# Autodesk Inventor assembly: A2017_T3_01
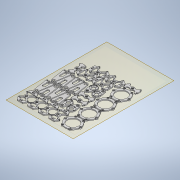
[picture p0: Inventor's stored thumbnail of the model, 180x180]
Saved by Autodesk Inventor 2020 (Build 240168000, 168)
## iProperties
Created: 2021-08-27
Part Number: A2017_T3_01
Document SubType Name: Assembly
Designer: Masato
Author: Masato
## Documents named in this file (7)
- C:\Users\naoki\Documents\Inventor\CitBrains\git_clone\SUSTAINA_ver1_0\A2017_T5_02(sustaina_op)\SUSTAINA-OP\Cam\A2017_T3_01.iam
- C:\Users\naoki\Documents\Inventor\CitBrains\git_clone\SUSTAINA_ver1_0\A2017_T5_02(sustaina_op)\SUSTAINA-OP\Cam\DisposableBoard.ipt
- C:\Users\naoki\Documents\Inventor\CitBrains\git_clone\SUSTAINA_ver1_0\A2017_T5_02(sustaina_op)\SUSTAINA-OP\LowerBody\Leg_joit\Leg_joint_roll_frame.ipt
- C:\Users\naoki\Documents\Inventor\CitBrains\git_clone\SUSTAINA_ver1_0\A2017_T5_02(sustaina_op)\SUSTAINA-OP\LowerBody\Leg_joit\Leg_joint_slider_frame.ipt
- C:\Users\naoki\Documents\Inventor\CitBrains\git_clone\SUSTAINA_ver1_0\A2017_T5_02(sustaina_op)\SUSTAINA-OP\LowerBody\Slider_crank\Slider_crank_horn.ipt
- C:\Users\naoki\Documents\Inventor\CitBrains\git_clone\SUSTAINA_ver1_0\A2017_T5_02(sustaina_op)\SUSTAINA-OP\LowerBody\Ankle\Ankle_front_frame.ipt
- C:\Users\naoki\Documents\Inventor\CitBrains\git_clone\SUSTAINA_ver1_0\A2017_T5_02(sustaina_op)\SUSTAINA-OP\UpperBody\Trunk\CrossRollerBearing\Outer_flange.ipt
## Components (30 placed, 6 different names)
1. DisposableBoard:1 — メイト:2, メイト:1, フラッシュ:1, フラッシュ:2, フラッシュ:12, 正接:1, フラッシュ:13, 角度:1, メイト:8, 正接:8, 角度:2, メイト:10, メイト:11, メイト:12, メイト:13, 角度:3, メイト:19, メイト:21, 角度:4
2. Outer_flange:1 — フラッシュ:7
3. Leg_joint_roll_frame:6 — メイト:12, メイト:15, メイト:16, メイト:17
4. Leg_joint_roll_frame:7 — メイト:10, 正接:10, 正接:11, 角度:3, メイト:14, フラッシュ:14, メイト:15, メイト:18
5. Leg_joint_roll_frame:8 — メイト:13, メイト:14, フラッシュ:14, メイト:16, 正接:12
6. Leg_joint_roll_frame:9 — メイト:11, メイト:17, メイト:18
7. Ankle_front_frame:3 — メイト:21, 正接:13, 正接:14, 角度:4
8. Ankle_front_frame:4 — メイト:19, メイト:20, 正接:12
9. Leg_joint_roll_frame:1 — フラッシュ:3, フラッシュ:4, フラッシュ:5, フラッシュ:10, フラッシュ:12, 正接:1, 正接:2, メイト:8
10. Leg_joint_roll_frame:3
11. Leg_joint_roll_frame:4
12. Leg_joint_roll_frame:5 — 正接:4, 正接:5, 正接:7
13. Leg_joint_slider_frame:1 — フラッシュ:6, フラッシュ:7, フラッシュ:13, 正接:2, メイト:5, 正接:3
14. Leg_joint_slider_frame:2 — フラッシュ:5, フラッシュ:6, メイト:5, 正接:3
15. Leg_joint_slider_frame:3 — メイト:20
16. Leg_joint_slider_frame:4
17. Leg_joint_slider_frame:5
18. Leg_joint_slider_frame:6 — メイト:7
19. Leg_joint_slider_frame:7
20. Leg_joint_slider_frame:8 — メイト:9
21. Outer_flange:2 — フラッシュ:9, 角度:1, 正接:7, 正接:8
22. Outer_flange:3
23. Outer_flange:4
24. Outer_flange:5 — 正接:13, 正接:14
25. Ankle_front_frame:1 — フラッシュ:10, 角度:2, 正接:9
26. Ankle_front_frame:2 — メイト:9
27. Slider_crank_horn:1 — フラッシュ:3, メイト:6, 正接:5
28. Slider_crank_horn:2 — フラッシュ:4, フラッシュ:9, メイト:6, 正接:4, メイト:7, 正接:9
29. Slider_crank_horn:3 — 正接:11
30. Slider_crank_horn:4 — 正接:10
## Component patterns: (4 elements, first: Leg_joint_roll_frame:1), (4 elements, first: Leg_joint_slider_frame:1 + Leg_joint_slider_frame:2), (4 elements, first: Outer_flange:2), (2 elements, first: Ankle_front_frame:1), (2 elements, first: Slider_crank_horn:1 + Slider_crank_horn:2)
## Relationships (48: Mate 19, Tangent 13, Flush 12, Angle 4)
- メイト:2 [Mate]: DisposableBoard:1
- メイト:1 [Mate]: DisposableBoard:1
- フラッシュ:1 [Flush]: DisposableBoard:1
- フラッシュ:2 [Flush]: DisposableBoard:1
- フラッシュ:3 [Flush]: Leg_joint_roll_frame:1 ↔ Slider_crank_horn:1
- フラッシュ:4 [Flush]: Leg_joint_roll_frame:1 ↔ Slider_crank_horn:2
- フラッシュ:5 [Flush]: Leg_joint_roll_frame:1 ↔ Leg_joint_slider_frame:2
- フラッシュ:6 [Flush]: Leg_joint_slider_frame:1 ↔ Leg_joint_slider_frame:2
- フラッシュ:7 [Flush]: Outer_flange:1 ↔ Leg_joint_slider_frame:1
- フラッシュ:9 [Flush]: Outer_flange:2 ↔ Slider_crank_horn:2
- フラッシュ:10 [Flush]: Leg_joint_roll_frame:1 ↔ Ankle_front_frame:1
- フラッシュ:12 [Flush] (2 mm): DisposableBoard:1 ↔ Leg_joint_roll_frame:1
- 正接:1 [Tangent] (2 mm): DisposableBoard:1 ↔ Leg_joint_roll_frame:1
- フラッシュ:13 [Flush] (2 mm): DisposableBoard:1 ↔ Leg_joint_slider_frame:1
- 正接:2 [Tangent] (2.5 mm): Leg_joint_roll_frame:1 ↔ Leg_joint_slider_frame:1
- メイト:5 [Mate] (2.5 mm): Leg_joint_slider_frame:1 ↔ Leg_joint_slider_frame:2
- 正接:3 [Tangent]: Leg_joint_slider_frame:1 ↔ Leg_joint_slider_frame:2
- メイト:6 [Mate] (2.5 mm): Slider_crank_horn:1 ↔ Slider_crank_horn:2
- 正接:4 [Tangent] (2.5 mm): Leg_joint_roll_frame:5 ↔ Slider_crank_horn:2
- 正接:5 [Tangent] (2.5 mm): Leg_joint_roll_frame:5 ↔ Slider_crank_horn:1
- メイト:7 [Mate] (2.5 mm): Leg_joint_slider_frame:6 ↔ Slider_crank_horn:2
- 角度:1 [Angle] (30 deg): DisposableBoard:1 ↔ Outer_flange:2
- メイト:8 [Mate]: DisposableBoard:1 ↔ Leg_joint_roll_frame:1
- 正接:7 [Tangent] (1 mm): Leg_joint_roll_frame:5 ↔ Outer_flange:2
- 正接:8 [Tangent] (2 mm): DisposableBoard:1 ↔ Outer_flange:2
- 角度:2 [Angle] (0 deg): DisposableBoard:1 ↔ Ankle_front_frame:1
- メイト:9 [Mate] (2.5 mm): Leg_joint_slider_frame:8 ↔ Ankle_front_frame:2
- 正接:9 [Tangent] (2.5 mm): Ankle_front_frame:1 ↔ Slider_crank_horn:2
- メイト:10 [Mate]: DisposableBoard:1 ↔ Leg_joint_roll_frame:7
- メイト:11 [Mate]: DisposableBoard:1 ↔ Leg_joint_roll_frame:9
- メイト:12 [Mate]: DisposableBoard:1 ↔ Leg_joint_roll_frame:6
- メイト:13 [Mate]: DisposableBoard:1 ↔ Leg_joint_roll_frame:8
- 正接:10 [Tangent] (2.5 mm): Leg_joint_roll_frame:7 ↔ Slider_crank_horn:4
- 正接:11 [Tangent] (2.5 mm): Leg_joint_roll_frame:7 ↔ Slider_crank_horn:3
- 角度:3 [Angle] (-90 deg): DisposableBoard:1 ↔ Leg_joint_roll_frame:7
- メイト:14 [Mate] (2.5 mm): Leg_joint_roll_frame:7 ↔ Leg_joint_roll_frame:8
- フラッシュ:14 [Flush]: Leg_joint_roll_frame:7 ↔ Leg_joint_roll_frame:8
- メイト:15 [Mate] (2.5 mm): Leg_joint_roll_frame:6 ↔ Leg_joint_roll_frame:7
- メイト:16 [Mate] (2.5 mm): Leg_joint_roll_frame:6 ↔ Leg_joint_roll_frame:8
- メイト:17 [Mate] (2.5 mm): Leg_joint_roll_frame:6 ↔ Leg_joint_roll_frame:9
- メイト:18 [Mate] (2.5 mm): Leg_joint_roll_frame:7 ↔ Leg_joint_roll_frame:9
- メイト:19 [Mate]: DisposableBoard:1 ↔ Ankle_front_frame:4
- メイト:20 [Mate] (2.5 mm): Ankle_front_frame:4 ↔ Leg_joint_slider_frame:3
- 正接:12 [Tangent] (2.5 mm): Leg_joint_roll_frame:8 ↔ Ankle_front_frame:4
- メイト:21 [Mate]: DisposableBoard:1 ↔ Ankle_front_frame:3
- 正接:13 [Tangent] (2.5 mm): Ankle_front_frame:3 ↔ Outer_flange:5
- 正接:14 [Tangent] (2.5 mm): Ankle_front_frame:3 ↔ Outer_flange:5
- 角度:4 [Angle] (180 deg): DisposableBoard:1 ↔ Ankle_front_frame:3
